# Autodesk Inventor assembly: T-ESD-4
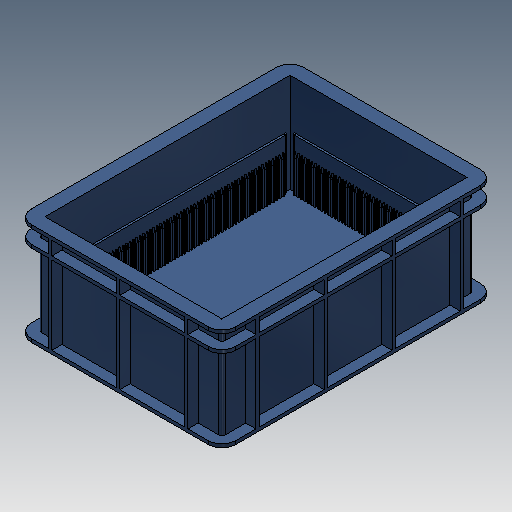
[picture p0: Inventor's stored thumbnail of the model, 512x512]
Saved by Autodesk Inventor 2018.3 (Build 223284000, 284)
## iProperties
Created: 2004-11-23
Part Number: T-ESD-4
Document SubType Name: Assembly
Designer: Autodesk, Inc.
Manufacturer: Standard
Standards Organization: Custom
Mass: 2161.22 g
Surface Area: 9822.36 cm^2
Volume: 2161.22 cm^3
Density: 1 g/cm^3
CAGE: 1LJX3
Dept. ID: Product Design
Description #2: ---
Finish #1: ---
Finish #2: ---
Material ID: ---
Project Number: ---
Author: Autodesk, Inc.
## Documents named in this file (4)
- C:\AVAInvAPI\Workspace\Test Station\Components\Standard Tote.iam
- C:\AVAInvAPI\Workspace\Test Station\Components\Tote Base.ipt
- C:\AVAInvAPI\Workspace\Test Station\Components\Slots Part.ipt
- C:\AVAInvAPI\Workspace\Test Station\Components\Slots Part 2.ipt
## Components (5 placed, 3 different names)
1. Tote Base:1 — Angle:1, Flush:1, Mate:2, Mate:3, Flush:3, Mate:6, Mate:8, Mate:5
2. Slots Part:1 — Mate:3, Flush:2
3. Slots Part:2 — Flush:1, Mate:2, Flush:2
4. Slots Part 2:1 — Flush:3, Mate:6, Flush:4, Mate:5
5. Slots Part 2:2 — Mate:8, Flush:4
## Relationships (11: Mate 6, Flush 4, Angle 1)
- Angle:1 (0 deg): Tote Base:1
- Flush:1: Tote Base:1 ↔ Slots Part:2
- Mate:2: Tote Base:1 ↔ Slots Part:2
- Mate:3: Tote Base:1 ↔ Slots Part:1
- Flush:2: Slots Part:1 ↔ Slots Part:2
- Flush:3: Tote Base:1 ↔ Slots Part 2:1
- Mate:6: Tote Base:1 ↔ Slots Part 2:1
- Mate:8: Tote Base:1 ↔ Slots Part 2:2
- Flush:4: Slots Part 2:1 ↔ Slots Part 2:2
- Mate:5: Tote Base:1 ↔ Slots Part 2:1
- [Mate]: Tote Base:1 ↔ Slots Part:2
